# Autodesk Inventor assembly: Xgantry_CableChain_top_connector_FULL
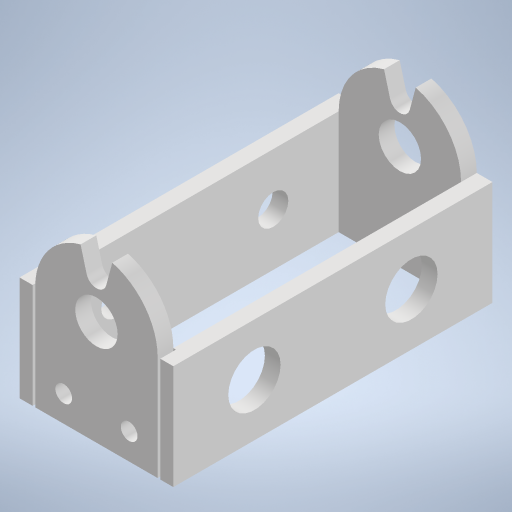
[picture p0: Inventor's stored thumbnail of the model, 512x512]
Saved by Autodesk Inventor 2023 (Build 270158000, 158)
## iProperties
Created: 2023-01-08
Part Number: Xgantry_CableChain_top_connector_FULL
Document SubType Name: Assembly
Designer: a laptop
Author: a laptop
## Documents named in this file (3)
- C:\Users\a laptop\Desktop\CNC_Project\Xgantry_CableChain_top_connector_FULL.iam
- C:\Users\a laptop\Desktop\CNC_Project\Xgantry_CableChain_top_connector.ipt
- C:\Users\a laptop\Desktop\CNC_Project\Xgantry_CableChain_top_connector_p2.ipt
## Components (2 placed, 2 different names)
1. Xgantry_CableChain_top_connector:1 — Mate:1, Mate:2, Mate:3
2. Xgantry_CableChain_top_connector_p2:1 — Mate:1, Mate:2, Mate:3
## Relationships (3: Mate 3)
- Mate:1: Xgantry_CableChain_top_connector:1 ↔ Xgantry_CableChain_top_connector_p2:1
- Mate:2: Xgantry_CableChain_top_connector:1 ↔ Xgantry_CableChain_top_connector_p2:1
- Mate:3: Xgantry_CableChain_top_connector:1 ↔ Xgantry_CableChain_top_connector_p2:1
